# Autodesk Inventor assembly: POM_T5_33
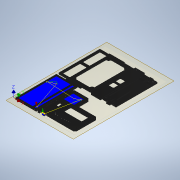
[picture p0: Inventor's stored thumbnail of the model, 180x180]
Saved by Autodesk Inventor 2020 (Build 240168000, 168)
## iProperties
Created: 2021-08-27
Part Number: POM_T5_33
Document SubType Name: Assembly
Designer: Masato
Author: Masato
## Documents named in this file (7)
- D:\GitHub\inventor\SUSTAINA-OP\Cam\POM_T5_33.iam
- D:\GitHub\inventor\SUSTAINA-OP\Cam\DisposableBoard.ipt
- D:\GitHub\inventor\SUSTAINA-OP\UpperBody\Cockpit\Cockpit_circuit_board_frame.ipt
- D:\GitHub\inventor\SUSTAINA-OP\UpperBody\Cockpit\Cockpit_top_frame.ipt
- D:\GitHub\inventor\SUSTAINA-OP\UpperBody\Cockpit\Cockpit_front_frame.ipt
- D:\GitHub\inventor\SUSTAINA-OP\UpperBody\Cockpit\Cockpit_side_frame.ipt
- D:\GitHub\inventor\SUSTAINA-OP\UpperBody\Cockpit\Cockpit_battery_bottom_frame.ipt
## Components (6 placed, 6 different names)
1. DisposableBoard:1 — メイト:2, メイト:1, フラッシュ:1, フラッシュ:2, メイト:22, メイト:24, メイト:28, フラッシュ:7, フラッシュ:8, メイト:36, メイト:42
2. Cockpit_circuit_board_frame:1 — メイト:28, フラッシュ:9, メイト:41, フラッシュ:12, フラッシュ:13
3. Cockpit_top_frame:1 — メイト:22, メイト:27, メイト:41, フラッシュ:13, メイト:43
4. Cockpit_front_frame:1 — メイト:24, メイト:27, フラッシュ:7, フラッシュ:8, フラッシュ:9, フラッシュ:11, メイト:37
5. Cockpit_side_frame:1 — メイト:36, フラッシュ:11, メイト:37
6. Cockpit_battery_bottom_frame:1 — メイト:42, フラッシュ:12, メイト:43
## Relationships (19: Mate 11, Flush 8)
- メイト:2 [Mate]: DisposableBoard:1
- メイト:1 [Mate]: DisposableBoard:1
- フラッシュ:1 [Flush]: DisposableBoard:1
- フラッシュ:2 [Flush]: DisposableBoard:1
- メイト:22 [Mate]: DisposableBoard:1 ↔ Cockpit_top_frame:1
- メイト:24 [Mate]: DisposableBoard:1 ↔ Cockpit_front_frame:1
- メイト:27 [Mate] (2.5 mm): Cockpit_top_frame:1 ↔ Cockpit_front_frame:1
- メイト:28 [Mate]: DisposableBoard:1 ↔ Cockpit_circuit_board_frame:1
- フラッシュ:7 [Flush] (2.5 mm): DisposableBoard:1 ↔ Cockpit_front_frame:1
- フラッシュ:8 [Flush] (2.5 mm): DisposableBoard:1 ↔ Cockpit_front_frame:1
- フラッシュ:9 [Flush]: Cockpit_circuit_board_frame:1 ↔ Cockpit_front_frame:1
- メイト:36 [Mate]: DisposableBoard:1 ↔ Cockpit_side_frame:1
- フラッシュ:11 [Flush]: Cockpit_front_frame:1 ↔ Cockpit_side_frame:1
- メイト:37 [Mate] (2.5 mm): Cockpit_front_frame:1 ↔ Cockpit_side_frame:1
- メイト:41 [Mate] (2.5 mm): Cockpit_circuit_board_frame:1 ↔ Cockpit_top_frame:1
- メイト:42 [Mate]: DisposableBoard:1 ↔ Cockpit_battery_bottom_frame:1
- フラッシュ:12 [Flush]: Cockpit_circuit_board_frame:1 ↔ Cockpit_battery_bottom_frame:1
- フラッシュ:13 [Flush]: Cockpit_circuit_board_frame:1 ↔ Cockpit_top_frame:1
- メイト:43 [Mate] (2.5 mm): Cockpit_top_frame:1 ↔ Cockpit_battery_bottom_frame:1
